# Autodesk Inventor assembly: Assembly1
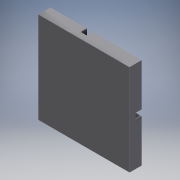
[picture p0: Inventor's stored thumbnail of the model, 180x180]
Saved by Autodesk Inventor 2019 (Build 230136000, 136)
## iProperties
Created: 2021-08-31
Part Number: Assembly1
Document SubType Name: Assembly
Designer: zachm
Author: zachm
## Documents named in this file (9)
- C:\Users\zachm\OneDrive\Documents\University\Year 4\700 Research Project\Junctions\Assembly1.iam
- C:\Users\zachm\OneDrive\Documents\University\Year 4\700 Research Project\Junctions\board.ipt
- C:\Users\zachm\OneDrive\Documents\University\Year 4\700 Research Project\Junctions\core_b_termination.ipt
- C:\Users\zachm\OneDrive\Documents\University\Year 4\700 Research Project\Junctions\core_b_through.ipt
- C:\Users\zachm\OneDrive\Documents\University\Year 4\700 Research Project\Junctions\core_r_termination.ipt
- C:\Users\zachm\OneDrive\Documents\University\Year 4\700 Research Project\Junctions\core_r_through.ipt
- C:\Users\zachm\OneDrive\Documents\University\Year 4\700 Research Project\Junctions\core_y_termination.ipt
- C:\Users\zachm\OneDrive\Documents\University\Year 4\700 Research Project\Junctions\core_y_through.ipt
- C:\Users\zachm\OneDrive\Documents\University\Year 4\700 Research Project\Junctions\IPC_35.ipt
## Components (10 placed, 8 different names)
1. board:1 — Tangent:1, Tangent:2, Mate:1, Tangent:3, Mate:2, Tangent:5, Mate:3, Tangent:7, Mate:4, Tangent:8, Tangent:9, Mate:5, Tangent:11, Flush:1, Tangent:12, Mate:6, Mate:7, Flush:2, Flush:3
2. core_b_termination:1 — Tangent:7, Mate:4, Tangent:8, Tangent:10
3. core_b_through:1 — Tangent:1, Tangent:2, Mate:1, Tangent:4, Tangent:13
4. core_r_termination:1 — Tangent:11, Flush:1, Tangent:12, Tangent:14
5. core_r_through:1 — Tangent:3, Mate:2, Tangent:4, Tangent:6, Tangent:15
6. core_y_termination:1 — Tangent:9, Tangent:10, Mate:5, Tangent:16
7. core_y_through:1 — Tangent:5, Mate:3, Tangent:6, Tangent:17
8. IPC_35:1 — Mate:6, Tangent:13, Mate:7
9. IPC_35:2 — Flush:3, Tangent:16, Tangent:17
10. IPC_35:3 — Tangent:14, Flush:2, Tangent:15
## Relationships (27: Tangent 17, Mate 7, Flush 3)
- Tangent:1: board:1 ↔ core_b_through:1
- Tangent:2 (0.75 mm): board:1 ↔ core_b_through:1
- Mate:1 (-2.5 mm): board:1 ↔ core_b_through:1
- Tangent:3: board:1 ↔ core_r_through:1
- Mate:2 (-2.5 mm): board:1 ↔ core_r_through:1
- Tangent:4 (0.75 mm): core_b_through:1 ↔ core_r_through:1
- Tangent:5: board:1 ↔ core_y_through:1
- Mate:3 (-2.5 mm): board:1 ↔ core_y_through:1
- Tangent:6 (0.75 mm): core_r_through:1 ↔ core_y_through:1
- Tangent:7: board:1 ↔ core_b_termination:1
- Mate:4: board:1 ↔ core_b_termination:1
- Tangent:8 (0.75 mm): board:1 ↔ core_b_termination:1
- Tangent:9: board:1 ↔ core_y_termination:1
- Tangent:10 (8.5 mm): core_b_termination:1 ↔ core_y_termination:1
- Mate:5: board:1 ↔ core_y_termination:1
- Tangent:11: board:1 ↔ core_r_termination:1
- Flush:1: board:1 ↔ core_r_termination:1
- Tangent:12 (0.75 mm): board:1 ↔ core_r_termination:1
- Mate:6: board:1 ↔ IPC_35:1
- Tangent:13: core_b_through:1 ↔ IPC_35:1
- Mate:7: board:1 ↔ IPC_35:1
- Tangent:14: core_r_termination:1 ↔ IPC_35:3
- Flush:2 (5 mm): board:1 ↔ IPC_35:3
- Tangent:15: core_r_through:1 ↔ IPC_35:3
- Flush:3 (-5 mm): board:1 ↔ IPC_35:2
- Tangent:16: core_y_termination:1 ↔ IPC_35:2
- Tangent:17: core_y_through:1 ↔ IPC_35:2
